# Autodesk Inventor assembly: 12020 Motorized Slider
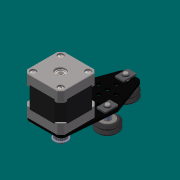
[picture p0: Inventor's stored thumbnail of the model, 180x180]
Saved by Autodesk Inventor 2016 (Build 200138000, 138)
## iProperties
Created: 2015-06-02
Part Number: 12020 Motorized Slider
Document SubType Name: Assembly
Designer: Sawaiz Syed
Author: Sawaiz Syed
## Documents named in this file (6)
- C:\Users\Sawaiz\Documents\data\projects\cncBlackBox\yAxis\slider\motorizedSlider.iam
- C:\Users\Sawaiz\Documents\data\projects\cncBlackBox\vWheel\vWheelSpacerTNut.iam
- C:\Users\Sawaiz\Documents\data\projects\cncBlackBox\vWheel\vWheelEccentricTNut.iam
- C:\Users\Sawaiz\Documents\data\projects\cncBlackBox\yAxis\slider\motorizedSliderPlate.ipt
- C:\Users\Sawaiz\Documents\data\projects\cncBlackBox\nema17Stepper\nema17t5.iam
- C:\Users\Sawaiz\Documents\data\projects\cncBlackBox\hardware\m3x8.ipt
## Components (9 placed, 5 different names)
1. motorizedSliderPlate:1 — Mate:1, Mate:2, Mate:3, Mate:4, Angle:4, Mate:9, Mate:11, Angle:7, Mate:15
2. vWheelSpacerTNut:1 [sub-assembly] — Mate:2, Flush:1, Angle:6, Flush:7
3. vWheelEccentricTNut:1 [sub-assembly] — Mate:3, Flush:2, Angle:5, Angle:7, Flush:6, Flush:7
4. vWheelSpacerTNut:2 [sub-assembly] — Mate:1, Flush:1, Flush:2, Mate:4, Angle:5, Angle:6, Flush:6
5. nema17t5:1 [sub-assembly] — Mate:8, Angle:4, Mate:9, Mate:11, Mate:12, Mate:13, Mate:14
6. m3x8:1 — Mate:12, Flush:3, Flush:4
7. m3x8:2 — Mate:14, Flush:5
8. m3x8:3 — Mate:13, Flush:4, Flush:5, Mate:15
9. m3x8:4 — Mate:8, Flush:3
## Relationships (22: Mate 11, Flush 7, Angle 4)
- Mate:1: motorizedSliderPlate:1 ↔ vWheelSpacerTNut:2
- Mate:2: motorizedSliderPlate:1 ↔ vWheelSpacerTNut:1
- Mate:3: motorizedSliderPlate:1 ↔ vWheelEccentricTNut:1
- Flush:1: vWheelSpacerTNut:1 ↔ vWheelSpacerTNut:2
- Flush:2: vWheelEccentricTNut:1 ↔ vWheelSpacerTNut:2
- Mate:4: motorizedSliderPlate:1 ↔ vWheelSpacerTNut:2
- Mate:8: nema17t5:1 ↔ m3x8:4
- Angle:4 (0 deg): motorizedSliderPlate:1 ↔ nema17t5:1
- Mate:9: motorizedSliderPlate:1 ↔ nema17t5:1
- Mate:11: motorizedSliderPlate:1 ↔ nema17t5:1
- Angle:5 (0 deg): vWheelEccentricTNut:1 ↔ vWheelSpacerTNut:2
- Angle:6 (0 deg): vWheelSpacerTNut:1 ↔ vWheelSpacerTNut:2
- Angle:7 (0 deg): motorizedSliderPlate:1 ↔ vWheelEccentricTNut:1
- Mate:12: nema17t5:1 ↔ m3x8:1
- Mate:13: nema17t5:1 ↔ m3x8:3
- Mate:14: nema17t5:1 ↔ m3x8:2
- Flush:3: m3x8:1 ↔ m3x8:4
- Flush:4: m3x8:1 ↔ m3x8:3
- Flush:5: m3x8:2 ↔ m3x8:3
- Mate:15: motorizedSliderPlate:1 ↔ m3x8:3
- Flush:6: vWheelEccentricTNut:1 ↔ vWheelSpacerTNut:2
- Flush:7: vWheelSpacerTNut:1 ↔ vWheelEccentricTNut:1
